# Autodesk Inventor assembly: OmniWheel
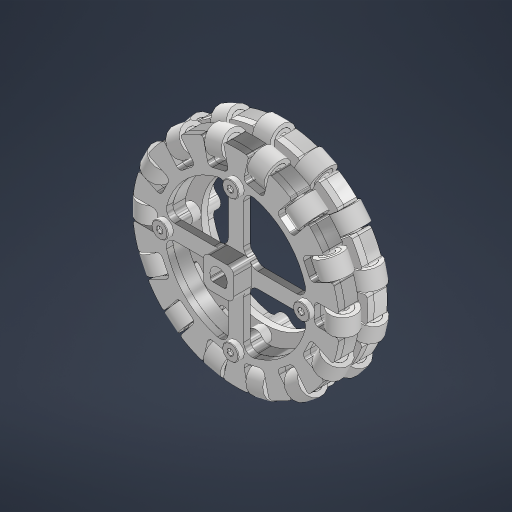
[picture p0: Inventor's stored thumbnail of the model, 512x512]
Saved by Autodesk Inventor 2024.2 (Build 282272000, 272)
## iProperties
Created: 2023-12-20
Part Number: OmniWheel
Document SubType Name: Assembly
Designer: Hanaoka
Author: Hanaoka
## Documents named in this file (7)
- G:\共有ドライブ\reRo\05_個人\hanaoka\inventor\DriveUnit\OmniWheel.iam
- G:\共有ドライブ\reRo\05_個人\hanaoka\inventor\DriveUnit\OmniFrame_B.ipt
- G:\共有ドライブ\reRo\05_個人\hanaoka\inventor\DriveUnit\SideWheel.iam
- G:\共有ドライブ\reRo\05_個人\hanaoka\inventor\DriveUnit\OmniFrame_A.ipt
- G:\共有ドライブ\reRo\05_個人\hanaoka\inventor\DriveUnit\OmniFrame_D.ipt
- G:\共有ドライブ\reRo\05_個人\hanaoka\inventor\DriveUnit\OmniFrame_C.ipt
- G:\共有ドライブ\reRo\05_個人\hanaoka\inventor\Screw\M2xL6\M2x6.ipt
## Components (36 placed, 6 different names)
1. OmniFrame_B:1 — メイト:2, メイト:3, メイト:4, メイト:5, 正接:2, 正接:3, 挿入:4, 挿入:12
2. OmniFrame_A:1 — フラッシュ:1, 正接:1, メイト:1, メイト:2, メイト:3, メイト:4, 挿入:8, 挿入:9, 挿入:10, 挿入:11
3. OmniFrame_D:1 — 挿入:13, 挿入:14, 正接:4, メイト:6
4. OmniFrame_C:1 — 挿入:4, 挿入:12, 挿入:13, 挿入:14, 正接:5
5. M2x6:1 — 挿入:11
6. M2x6:2 — 挿入:10
7. M2x6:3 — 挿入:9
8. M2x6:4 — 挿入:8
9. SideWheel:1 [sub-assembly] — メイト:5, 正接:2, 正接:3
10. SideWheel:2 [sub-assembly]
11. SideWheel:3 [sub-assembly]
12. SideWheel:4 [sub-assembly]
13. SideWheel:5 [sub-assembly]
14. SideWheel:6 [sub-assembly]
15. SideWheel:7 [sub-assembly]
16. SideWheel:8 [sub-assembly]
17. SideWheel:9 [sub-assembly]
18. SideWheel:10 [sub-assembly]
19. SideWheel:11 [sub-assembly]
20. SideWheel:12 [sub-assembly]
21. SideWheel:13 [sub-assembly]
22. SideWheel:14 [sub-assembly]
23. SideWheel:15 [sub-assembly] — 正接:4, メイト:6, 正接:5
24. SideWheel:16 [sub-assembly]
25. SideWheel:17 [sub-assembly]
26. SideWheel:18 [sub-assembly]
27. SideWheel:19 [sub-assembly]
28. SideWheel:20 [sub-assembly]
29. SideWheel:21 [sub-assembly]
30. SideWheel:22 [sub-assembly]
31. SideWheel:23 [sub-assembly]
32. SideWheel:24 [sub-assembly]
33. SideWheel:25 [sub-assembly]
34. SideWheel:26 [sub-assembly]
35. SideWheel:27 [sub-assembly]
36. SideWheel:28 [sub-assembly]
## Component patterns: (14 elements, first: SideWheel:1), (14 elements, first: SideWheel:15)
## Relationships (20: Insert 8, Mate 6, Tangent 5, Flush 1)
- フラッシュ:1 [Flush]: OmniFrame_A:1
- 正接:1 [Tangent]: OmniFrame_A:1
- メイト:1 [Mate] (6 mm): OmniFrame_A:1
- メイト:2 [Mate]: OmniFrame_B:1 ↔ OmniFrame_A:1
- メイト:3 [Mate]: OmniFrame_B:1 ↔ OmniFrame_A:1
- メイト:4 [Mate]: OmniFrame_B:1 ↔ OmniFrame_A:1
- メイト:5 [Mate] (0.25 mm): OmniFrame_B:1 ↔ SideWheel:1
- 正接:2 [Tangent] (0.025 mm): OmniFrame_B:1 ↔ SideWheel:1
- 正接:3 [Tangent] (0.025 mm): OmniFrame_B:1 ↔ SideWheel:1
- 挿入:4 [Insert]: OmniFrame_B:1 ↔ OmniFrame_C:1
- 挿入:8 [Insert]: OmniFrame_A:1 ↔ M2x6:4
- 挿入:9 [Insert]: OmniFrame_A:1 ↔ M2x6:3
- 挿入:10 [Insert]: OmniFrame_A:1 ↔ M2x6:2
- 挿入:11 [Insert]: OmniFrame_A:1 ↔ M2x6:1
- 挿入:12 [Insert]: OmniFrame_B:1 ↔ OmniFrame_C:1
- 挿入:13 [Insert]: OmniFrame_D:1 ↔ OmniFrame_C:1
- 挿入:14 [Insert]: OmniFrame_D:1 ↔ OmniFrame_C:1
- 正接:4 [Tangent]: OmniFrame_D:1 ↔ SideWheel:15
- メイト:6 [Mate] (-0.5 mm): OmniFrame_D:1 ↔ SideWheel:15
- 正接:5 [Tangent]: OmniFrame_C:1 ↔ SideWheel:15
